# Autodesk Inventor assembly: assembly with all holes
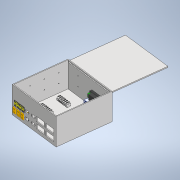
[picture p0: Inventor's stored thumbnail of the model, 180x180]
Saved by Autodesk Inventor 2020 (Build 240168000, 168)
## iProperties
Created: 2020-01-15
Part Number: assembly with all holes
Document SubType Name: Assembly
Designer: ColinP
Author: ColinP
## Documents named in this file (8)
- C:\Users\ColinP\Documents\Inventor\HeaterControlIQC\assembly with all holes.iam
- C:\Users\ColinP\Documents\Inventor\HeaterControlIQC\box but slightly bigger.ipt
- C:\Users\ColinP\Documents\Inventor\HeaterControlIQC\06AE2.ipt
- C:\Users\ColinP\Documents\Inventor\HeaterControlIQC\4300-0705.ipt
- C:\Users\ColinP\Documents\Inventor\HeaterControlIQC\User Library-Thermocouple_Submini Jack.ipt
- C:\Users\ColinP\Documents\Inventor\HeaterControlIQC\CUI_VSK-S5-5UA-T (1)\CUI_VSK-S5-5UA-T.iam
- C:\Users\ColinP\Documents\Inventor\HeaterControlIQC\OnShore_ES100006DS.ipt
- C:\Users\ColinP\Documents\Inventor\HeaterControlIQC\lid thin.ipt
## Components (14 placed, 7 different names)
1. box but slightly bigger:1 — Mate:1, Mate:4, Mate:5, Mate:6, Mate:7, Mate:8, Mate:9, Mate:10, Mate:11, Mate:12, Mate:13, Mate:14, Mate:15, Flush:1, Flush:2, Mate:16, Flush:3, Flush:4, Mate:17, Flush:5, Flush:6, Mate:18, Mate:22, Mate:23, Mate:24, Mate:25, Mate:26, Mate:27, Mate:28, Mate:29, Mate:30, Mate:34, Mate:35, Mate:38, Mate:39, Mate:40, Mate:41, Mate:42
2. 06AE2:1 — Mate:1, Mate:39, Mate:40
3. 4300-0705:1 — Flush:5, Flush:6, Mate:18
4. 4300-0705:2 — Flush:3, Flush:4, Mate:17
5. 4300-0705:3 — Flush:1, Flush:2, Mate:16
6. User Library-Thermocouple_Submini Jack:1 — Mate:10, Mate:11, Mate:12
7. User Library-Thermocouple_Submini Jack:2 — Mate:13, Mate:14, Mate:15
8. User Library-Thermocouple_Submini Jack:3 — Mate:7, Mate:8, Mate:9
9. User Library-Thermocouple_Submini Jack:4 — Mate:4, Mate:5, Mate:6
10. CUI_VSK-S5-5UA-T:1 [sub-assembly] — Mate:34, Mate:35, Mate:38
11. OnShore_ES100006DS:1 — Mate:25, Mate:29, Mate:30
12. OnShore_ES100006DS:2 — Mate:26, Mate:27, Mate:28
13. OnShore_ES100006DS:3 — Mate:22, Mate:23, Mate:24
14. lid thin:1 — Mate:41, Mate:42
## Relationships (38: Mate 32, Flush 6)
- Mate:1: box but slightly bigger:1 ↔ 06AE2:1
- Mate:4: box but slightly bigger:1 ↔ User Library-Thermocouple_Submini Jack:4
- Mate:5: box but slightly bigger:1 ↔ User Library-Thermocouple_Submini Jack:4
- Mate:6: box but slightly bigger:1 ↔ User Library-Thermocouple_Submini Jack:4
- Mate:7: box but slightly bigger:1 ↔ User Library-Thermocouple_Submini Jack:3
- Mate:8: box but slightly bigger:1 ↔ User Library-Thermocouple_Submini Jack:3
- Mate:9: box but slightly bigger:1 ↔ User Library-Thermocouple_Submini Jack:3
- Mate:10: box but slightly bigger:1 ↔ User Library-Thermocouple_Submini Jack:1
- Mate:11: box but slightly bigger:1 ↔ User Library-Thermocouple_Submini Jack:1
- Mate:12: box but slightly bigger:1 ↔ User Library-Thermocouple_Submini Jack:1
- Mate:13: box but slightly bigger:1 ↔ User Library-Thermocouple_Submini Jack:2
- Mate:14: box but slightly bigger:1 ↔ User Library-Thermocouple_Submini Jack:2
- Mate:15: box but slightly bigger:1 ↔ User Library-Thermocouple_Submini Jack:2
- Flush:1: box but slightly bigger:1 ↔ 4300-0705:3
- Flush:2: box but slightly bigger:1 ↔ 4300-0705:3
- Mate:16: box but slightly bigger:1 ↔ 4300-0705:3
- Flush:3: box but slightly bigger:1 ↔ 4300-0705:2
- Flush:4: box but slightly bigger:1 ↔ 4300-0705:2
- Mate:17: box but slightly bigger:1 ↔ 4300-0705:2
- Flush:5: box but slightly bigger:1 ↔ 4300-0705:1
- Flush:6: box but slightly bigger:1 ↔ 4300-0705:1
- Mate:18: box but slightly bigger:1 ↔ 4300-0705:1
- Mate:22: box but slightly bigger:1 ↔ OnShore_ES100006DS:3
- Mate:23: box but slightly bigger:1 ↔ OnShore_ES100006DS:3
- Mate:24: box but slightly bigger:1 ↔ OnShore_ES100006DS:3
- Mate:25: box but slightly bigger:1 ↔ OnShore_ES100006DS:1
- Mate:26: box but slightly bigger:1 ↔ OnShore_ES100006DS:2
- Mate:27: box but slightly bigger:1 ↔ OnShore_ES100006DS:2
- Mate:28: box but slightly bigger:1 ↔ OnShore_ES100006DS:2
- Mate:29: box but slightly bigger:1 ↔ OnShore_ES100006DS:1
- Mate:30: box but slightly bigger:1 ↔ OnShore_ES100006DS:1
- Mate:34: box but slightly bigger:1 ↔ CUI_VSK-S5-5UA-T:1
- Mate:35: box but slightly bigger:1 ↔ CUI_VSK-S5-5UA-T:1
- Mate:38: box but slightly bigger:1 ↔ CUI_VSK-S5-5UA-T:1
- Mate:39: box but slightly bigger:1 ↔ 06AE2:1
- Mate:40: box but slightly bigger:1 ↔ 06AE2:1
- Mate:41: box but slightly bigger:1 ↔ lid thin:1
- Mate:42: box but slightly bigger:1 ↔ lid thin:1
